# Autodesk Inventor assembly: Pins
(part 2 of 2)
- C:\Users\caleb\Desktop\Shared\Software\Hardware\ETL\modules\Tamale v2.0\module_r50\WS_AVSS.ipt
- C:\Users\caleb\Desktop\Shared\Software\Hardware\ETL\modules\Tamale v2.0\module_r50\WS_AVSS_1.ipt
- C:\Users\caleb\Desktop\Shared\Software\Hardware\ETL\modules\Tamale v2.0\module_r50\WS_AVSS_2.ipt
- C:\Users\caleb\Desktop\Shared\Software\Hardware\ETL\modules\Tamale v2.0\module_r50\WS_AVSS_3.ipt
- C:\Users\caleb\Desktop\Shared\Software\Hardware\ETL\modules\Tamale v2.0\module_r50\WS_AVSS8.ipt
- C:\Users\caleb\Desktop\Shared\Software\Hardware\ETL\modules\Tamale v2.0\module_r50\WS_AVSS8_1.ipt
- C:\Users\caleb\Desktop\Shared\Software\Hardware\ETL\modules\Tamale v2.0\module_r50\WS_AVSS8_2.ipt
- C:\Users\caleb\Desktop\Shared\Software\Hardware\ETL\modules\Tamale v2.0\module_r50\WS_AVSS8_3.ipt
- C:\Users\caleb\Desktop\Shared\Software\Hardware\ETL\modules\Tamale v2.0\module_r50\WS_DVDD.ipt
- C:\Users\caleb\Desktop\Shared\Software\Hardware\ETL\modules\Tamale v2.0\module_r50\WS_DVDD_1.ipt
- C:\Users\caleb\Desktop\Shared\Software\Hardware\ETL\modules\Tamale v2.0\module_r50\WS_DVDD_2.ipt
- C:\Users\caleb\Desktop\Shared\Software\Hardware\ETL\modules\Tamale v2.0\module_r50\WS_DVDD_3.ipt
- C:\Users\caleb\Desktop\Shared\Software\Hardware\ETL\modules\Tamale v2.0\module_r50\WS_DVDD10.ipt
- C:\Users\caleb\Desktop\Shared\Software\Hardware\ETL\modules\Tamale v2.0\module_r50\WS_DVDD10_1.ipt
- C:\Users\caleb\Desktop\Shared\Software\Hardware\ETL\modules\Tamale v2.0\module_r50\WS_DVDD10_2.ipt
- C:\Users\caleb\Desktop\Shared\Software\Hardware\ETL\modules\Tamale v2.0\module_r50\WS_DVDD10_3.ipt
- C:\Users\caleb\Desktop\Shared\Software\Hardware\ETL\modules\Tamale v2.0\module_r50\WS_DVSS.ipt
- C:\Users\caleb\Desktop\Shared\Software\Hardware\ETL\modules\Tamale v2.0\module_r50\WS_DVSS_1.ipt
- C:\Users\caleb\Desktop\Shared\Software\Hardware\ETL\modules\Tamale v2.0\module_r50\WS_DVSS_2.ipt
- C:\Users\caleb\Desktop\Shared\Software\Hardware\ETL\modules\Tamale v2.0\module_r50\WS_DVSS_3.ipt
- C:\Users\caleb\Desktop\Shared\Software\Hardware\ETL\modules\Tamale v2.0\module_r50\WS_DVSS6.ipt
- C:\Users\caleb\Desktop\Shared\Software\Hardware\ETL\modules\Tamale v2.0\module_r50\WS_DVSS6_1.ipt
- C:\Users\caleb\Desktop\Shared\Software\Hardware\ETL\modules\Tamale v2.0\module_r50\WS_DVSS6_2.ipt
- C:\Users\caleb\Desktop\Shared\Software\Hardware\ETL\modules\Tamale v2.0\module_r50\WS_DVSS6_3.ipt
- C:\Users\caleb\Desktop\Shared\Software\Hardware\ETL\modules\Tamale v2.0\module_r50\WS_RSTN.ipt
- C:\Users\caleb\Desktop\Shared\Software\Hardware\ETL\modules\Tamale v2.0\module_r50\WS_RSTN_1.ipt
- C:\Users\caleb\Desktop\Shared\Software\Hardware\ETL\modules\Tamale v2.0\module_r50\WS_RSTN_2.ipt
- C:\Users\caleb\Desktop\Shared\Software\Hardware\ETL\modules\Tamale v2.0\module_r50\WS_RSTN_3.ipt
- C:\Users\caleb\Desktop\Shared\Software\Hardware\ETL\modules\Tamale v2.0\module_r50\WS_SCL.ipt
- C:\Users\caleb\Desktop\Shared\Software\Hardware\ETL\modules\Tamale v2.0\module_r50\WS_SCL_1.ipt
- C:\Users\caleb\Desktop\Shared\Software\Hardware\ETL\modules\Tamale v2.0\module_r50\WS_SCL_2.ipt
- C:\Users\caleb\Desktop\Shared\Software\Hardware\ETL\modules\Tamale v2.0\module_r50\WS_SCL_3.ipt
- C:\Users\caleb\Desktop\Shared\Software\Hardware\ETL\modules\Tamale v2.0\module_r50\WS_SDA.ipt
- C:\Users\caleb\Desktop\Shared\Software\Hardware\ETL\modules\Tamale v2.0\module_r50\WS_SDA_1.ipt
- C:\Users\caleb\Desktop\Shared\Software\Hardware\ETL\modules\Tamale v2.0\module_r50\WS_SDA_2.ipt
- C:\Users\caleb\Desktop\Shared\Software\Hardware\ETL\modules\Tamale v2.0\module_r50\WS_SDA_3.ipt
- C:\Users\caleb\Desktop\Shared\Software\Hardware\ETL\modules\Tamale v2.0\module_r50\WS_WR_EN.ipt
- C:\Users\caleb\Desktop\Shared\Software\Hardware\ETL\modules\Tamale v2.0\module_r50\WS_WR_EN_1.ipt
- C:\Users\caleb\Desktop\Shared\Software\Hardware\ETL\modules\Tamale v2.0\module_r50\WS_WR_EN_2.ipt
- C:\Users\caleb\Desktop\Shared\Software\Hardware\ETL\modules\Tamale v2.0\module_r50\WS_WR_EN_3.ipt
## Components (558 placed, 143 different names)
1. 1
2. 1:1
3. 1:2
4. 1:3
5. 1:4
6. 1:5
7. 1:6
8. 1:7
9. 1:8
10. 1:9
11. 1:10
12. 1:11
13. 1:12
14. 1:13
15. 1:14
16. 1:15
17. 1:16
18. 1:17
19. 1:18
20. 1:19
21. 1:20
22. 1:21
23. 1:22
24. 1:23
25. 1:24
26. 1:25
27. 1:26
28. 1:27
29. 1:28
30. 1:29
31. 1:30
32. 1:31
33. 1:32
34. 1:33
35. 1:34
36. 1:35
37. 1:36
38. 1:37
39. 1:38
40. 1:39
41. 1:40
42. 1:41
43. 1:42
44. 1:43
45. 1:44
46. 1:45
47. 1:46
48. 1:47
49. 1:48
50. 1:49
51. 1:50
52. 1:51
53. 1:52
54. 1:53
55. 1:54
56. 1:55
57. 1:56
58. 1:57
59. 1:58
60. 1:59
61. 1:60
62. 1:61
63. 1:62
64. 1:63
65. 1:64
66. 1:65
67. 1:66
68. 1:67
69. 1:68
70. 1:69
71. 1:70
72. 1:71
73. 1:72
74. 1:73
75. 1:74
76. 1:75
77. 1:76
78. 1:77
79. 1:78
80. 1:79
81. 1:80
82. 1:81
83. 1:82
84. 1:83
85. 1:84
86. 1:85
87. 1:86
88. 1:87
89. 1:88
90. 1:89
91. 1:90
92. 1:91
93. 1:92
94. 1:93
95. 1:94
96. 1:95
97. 1:96
98. 1:97
99. 1:98
100. 1:99
101. 1:100
102. 1:101
103. 1:102
104. 1:103
105. 1:104
106. 1:105
107. 1:106
108. 1:107
109. 1:108
110. 1:109
111. 1:110
112. 1:111
113. 1:112
114. 10
115. 11
116. 12
117. 13
118. 14
119. 15
120. 16
121. 17
122. 18
123. 19
124. 2
125. 2:1
126. 2:2
127. 2:3
128. 2:4
129. 2:5
130. 2:6
131. 2:7
132. 2:8
133. 2:9
134. 2:10
135. 2:11
136. 2:12
137. 2:13
138. 2:14
139. 2:15
140. 2:16
141. 2:17
142. 2:18
143. 2:19
144. 2:20
145. 2:21
146. 2:22
147. 2:23
148. 2:24
149. 2:25
150. 2:26
151. 2:27
152. 2:28
153. 2:29
154. 2:30
155. 2:31
156. 2:32
157. 2:33
158. 2:34
159. 2:35
160. 2:36
161. 2:37
162. 2:38
163. 2:39
164. 2:40
165. 2:41
166. 2:42
167. 2:43
168. 2:44
169. 2:45
170. 2:46
171. 2:47
172. 2:48
173. 2:49
174. 2:50
175. 2:51
176. 2:52
177. 2:53
178. 2:54
179. 2:55
180. 2:56
181. 2:57
182. 2:58
183. 2:59
184. 2:60
185. 2:61
186. 2:62
187. 2:63
188. 2:64
189. 2:65
190. 2:66
191. 2:67
192. 2:68
193. 2:69
194. 2:70
195. 2:71
196. 2:72
197. 2:73
198. 2:74
199. 2:75
200. 2:76
201. 2:77
202. 2:78
203. 2:79
204. 2:80
205. 2:81
206. 2:82
207. 2:83
208. 2:84
209. 2:85
210. 2:86
211. 2:87
212. 2:88
213. 2:89
214. 2:90
215. 2:91
216. 2:92
217. 2:93
218. 2:94
219. 2:95
220. 2:96
221. 2:97
222. 2:98
223. 2:99
224. 2:100
225. 2:101
226. 2:102
227. 2:103
228. 2:104
229. 2:105
230. 2:106
231. 2:107
232. 2:108
233. 2:109
234. 2:110
235. 2:111
236. 2:112
237. 20
238. 21
239. 22
240. 23
241. 24
242. 25
243. 26
244. 27
245. 28
246. 29
247. 3
248. 3:1
249. 3:2
250. 30
251. 31
252. 32
253. 33
254. 34
255. 35
256. 36
257. 37
258. 38
259. 39
260. 4
261. 40
262. 41
263. 42
264. 43
265. 44
266. 45
267. 46
268. 47
269. 48
270. 49
271. 5
272. 50
273. 51
274. 52
275. 53
276. 54
277. 55
278. 56
279. 57
280. 58
281. 59
282. 6
283. 60
284. 61
285. 62
286. 63
287. 64
288. 65
289. 66
290. 67
291. 68
292. 69
293. 7
294. 70
295. 71
296. 72
297. 73
298. 74
299. 75
300. 76
301. 77
302. 78
303. 8
304. 9
305. CLK1280_N
306. CLK1280_N:1
307. CLK1280_N:2
308. CLK1280_N:3
309. CLK1280_P
310. CLK1280_P:1
311. CLK1280_P:2
312. CLK1280_P:3
313. CLK40_N
314. CLK40_N:1
315. CLK40_N:2
316. CLK40_N:3
317. CLK40_P
318. CLK40_P:1
319. CLK40_P:2
320. CLK40_P:3
321. DOL_N
322. DOL_N:1
323. DOL_N:2
324. DOL_N:3
325. DOL_P
326. DOL_P:1
327. DOL_P:2
328. DOL_P:3
329. DOR_N
330. DOR_N:1
331. DOR_N:2
332. DOR_N:3
333. DOR_P
334. DOR_P:1
335. DOR_P:2
336. DOR_P:3
337. FCN
338. FCN:1
339. FCN:2
340. FCN:3
341. FCP
342. FCP:1
343. FCP:2
344. FCP:3
345. I2C_ADDR0
346. I2C_ADDR0:1
347. I2C_ADDR0:2
348. I2C_ADDR0:3
349. I2C_ADDR1
350. I2C_ADDR1:1
351. I2C_ADDR1:2
352. I2C_ADDR1:3
353. I2C_ADDR2
354. I2C_ADDR2:1
355. I2C_ADDR2:2
356. I2C_ADDR2:3
357. I2C_ADDR3
358. I2C_ADDR3:1
359. I2C_ADDR3:2
360. I2C_ADDR3:3
361. I2C_ADDR4
362. I2C_ADDR4:1
363. I2C_ADDR4:2
364. I2C_ADDR4:3
365. POWER1
366. POWER2
367. RSTN
368. RSTN:1
369. RSTN:2
370. RSTN:3
371. SCL
372. SCL:1
373. SCL:2
374. SCL:3
375. SDA
376. SDA:1
377. SDA:2
378. SDA:3
379. TP
380. TP:1
381. TP:2
382. TP:3
383. VDD_A
384. VDD_A:1
385. VDD_A:2
386. VDD_A:3
387. VDD_A1
388. VDD_A1:1
389. VDD_A1:2
390. VDD_A1:3
391. VDD_A12
392. VDD_A12:1
393. VDD_A12:2
394. VDD_A12:3
395. VDD_A5
396. VDD_A5:1
397. VDD_A5:2
398. VDD_A5:3
399. VDD_D
400. VDD_D:1
401. VDD_D:2
402. VDD_D:3
403. VDD_D11
404. VDD_D11:1
405. VDD_D11:2
406. VDD_D11:3
407. VDD_D15
408. VDD_D15:1
409. VDD_D15:2
410. VDD_D15:3
411. VDD_D20
412. VDD_D20:1
413. VDD_D20:2
414. VDD_D20:3
415. VDD_D21
416. VDD_D21:1
417. VDD_D21:2
418. VDD_D21:3
419. VDD_EFUSE
420. VDD_EFUSE:1
421. VDD_EFUSE:2
422. VDD_EFUSE:3
423. VP
424. VP:1
425. VP:2
426. VP:3
427. VREF
428. VREF:1
429. VREF:2
430. VREF:3
431. VSS_A
432. VSS_A:1
433. VSS_A:2
434. VSS_A:3
435. VSS_A2
436. VSS_A2:1
437. VSS_A2:2
438. VSS_A2:3
439. VSS_A22
440. VSS_A22:1
441. VSS_A22:2
442. VSS_A22:3
443. VSS_A3
444. VSS_A3:1
445. VSS_A3:2
446. VSS_A3:3
447. VSS_A4
448. VSS_A4:1
449. VSS_A4:2
450. VSS_A4:3
451. VSS_A9
452. VSS_A9:1
453. VSS_A9:2
454. VSS_A9:3
455. VSS_AO
456. VSS_AO:1
457. VSS_AO:2
458. VSS_AO:3
459. VSS_D
460. VSS_D:1
461. VSS_D:2
462. VSS_D:3
463. VSS_D13
464. VSS_D13:1
465. VSS_D13:2
466. VSS_D13:3
467. VSS_D14
468. VSS_D14:1
469. VSS_D14:2
470. VSS_D14:3
471. VSS_D16
472. VSS_D16:1
473. VSS_D16:2
474. VSS_D16:3
475. VSS_D17
476. VSS_D17:1
477. VSS_D17:2
478. VSS_D17:3
479. VSS_D18
480. VSS_D18:1
481. VSS_D18:2
482. VSS_D18:3
483. VSS_D19
484. VSS_D19:1
485. VSS_D19:2
486. VSS_D19:3
487. VTEMP
488. VTEMP:1
489. VTEMP:2
490. VTEMP:3
491. WS_ADDR0
492. WS_ADDR0:1
493. WS_ADDR0:2
494. WS_ADDR0:3
495. WS_ADDR1
496. WS_ADDR1:1
497. WS_ADDR1:2
498. WS_ADDR1:3
499. WS_ADDR2
500. WS_ADDR2:1
501. WS_ADDR2:2
502. WS_ADDR2:3
503. WS_ADDR3
504. WS_ADDR3:1
505. WS_ADDR3:2
506. WS_ADDR3:3
507. WS_ADDR4
508. WS_ADDR4:1
509. WS_ADDR4:2
510. WS_ADDR4:3
511. WS_AVDD
512. WS_AVDD:1
513. WS_AVDD:2
514. WS_AVDD:3
515. WS_AVDD7
516. WS_AVDD7:1
517. WS_AVDD7:2
518. WS_AVDD7:3
519. WS_AVSS
520. WS_AVSS:1
521. WS_AVSS:2
522. WS_AVSS:3
523. WS_AVSS8
524. WS_AVSS8:1
525. WS_AVSS8:2
526. WS_AVSS8:3
527. WS_DVDD
528. WS_DVDD:1
529. WS_DVDD:2
530. WS_DVDD:3
531. WS_DVDD10
532. WS_DVDD10:1
533. WS_DVDD10:2
534. WS_DVDD10:3
535. WS_DVSS
536. WS_DVSS:1
537. WS_DVSS:2
538. WS_DVSS:3
539. WS_DVSS6
540. WS_DVSS6:1
541. WS_DVSS6:2
542. WS_DVSS6:3
543. WS_RSTN
544. WS_RSTN:1
545. WS_RSTN:2
546. WS_RSTN:3
547. WS_SCL
548. WS_SCL:1
549. WS_SCL:2
550. WS_SCL:3
551. WS_SDA
552. WS_SDA:1
553. WS_SDA:2
554. WS_SDA:3
555. WS_WR_EN
556. WS_WR_EN:1
557. WS_WR_EN:2
558. WS_WR_EN:3
